# Autodesk Inventor assembly: Assembly Mount Rack
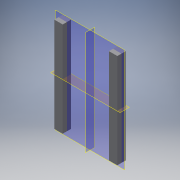
[picture p0: Inventor's stored thumbnail of the model, 180x180]
Saved by Autodesk Inventor 2019 (Build 230136000, 136)
## iProperties
Created: 2021-05-14
Part Number: Assembly Mount Rack
Document SubType Name: Assembly
Designer: Eric
Author: Eric
## Documents named in this file (3)
- C:\Users\Eric\Documents\! - Uni\Year 4\MENG-Robot-Fab-Project\Models\For_Optimiser\Static Parts Assembly\Assembly Mount Assembly\Assembly Mount Rack.iam
- C:\Users\Eric\Documents\! - Uni\Year 4\MENG-Robot-Fab-Project\Models\For_Optimiser\Static Parts Assembly\Assembly Mount Assembly\AssemblyMountRack_1.ipt
- C:\Users\Eric\Documents\! - Uni\Year 4\MENG-Robot-Fab-Project\Models\For_Optimiser\Static Parts Assembly\Assembly Mount Assembly\AssemblyMountRack_2.ipt
## Components (2 placed, 2 different names)
1. AssemblyMountRack_1:1 — Symmetry:1, Symmetry:2, Symmetry:3
2. AssemblyMountRack_2:1 — Symmetry:1, Symmetry:2, Symmetry:3
## Relationships (3: Symmetry 3)
- Symmetry:1: AssemblyMountRack_1:1 ↔ AssemblyMountRack_2:1
- Symmetry:2: AssemblyMountRack_1:1 ↔ AssemblyMountRack_2:1
- Symmetry:3: AssemblyMountRack_1:1 ↔ AssemblyMountRack_2:1
